# Autodesk Inventor assembly: CE-9.3.1
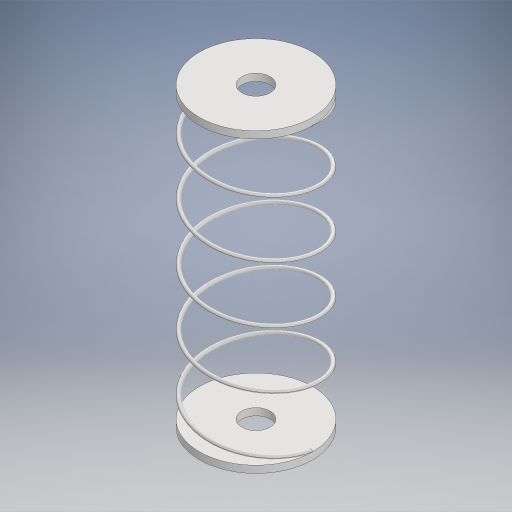
[picture p0: Inventor's stored thumbnail of the model, 512x512]
Saved by Autodesk Inventor 2024 (Build 280153000, 153)
## iProperties
Created: 2024-03-22
Part Number: CE-9.3.1
Document SubType Name: Assembly
Designer: Alex
Author: Alex
## Documents named in this file (3)
- C:\Shared\alex-bartella-schoolwork\4z03\Week 10\CE-9.3.1.iam
- C:\Shared\alex-bartella-schoolwork\4z03\Week 10\CE-9.3.1.ipt
- C:\Shared\alex-bartella-schoolwork\4z03\Week 10\CE-9.3.1-01-002.ipt
## Components (3 placed, 2 different names)
1. CE-9.3.1:1 — Flush:1, Flush:2, Flush:3, Driver:1, Flush:8
2. CE-9.3.1:2 — Flush:4, Flush:5, Driver:1
3. CE-9.3.1-01-002:1 — Flush:6, Flush:7, Flush:8
## Relationships (9: Flush 8, Mate 1)
- Flush:1: CE-9.3.1:1
- Flush:2: CE-9.3.1:1
- Flush:3: CE-9.3.1:1
- Flush:4: CE-9.3.1:2
- Flush:5: CE-9.3.1:2
- Driver:1 [Mate] (200 mm): CE-9.3.1:1 ↔ CE-9.3.1:2
- Flush:6: CE-9.3.1-01-002:1
- Flush:7: CE-9.3.1-01-002:1
- Flush:8: CE-9.3.1:1 ↔ CE-9.3.1-01-002:1
